# Autodesk Inventor assembly: wire_case-1
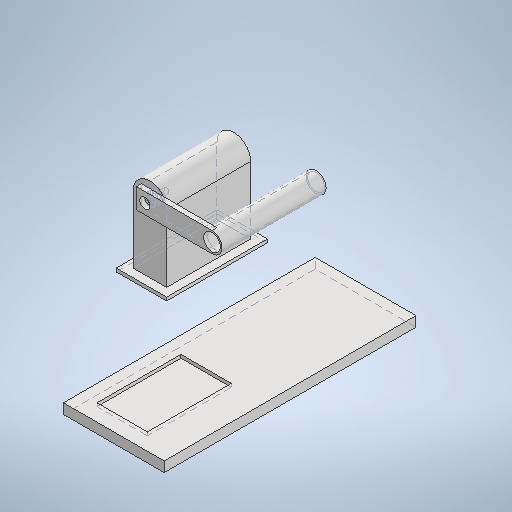
[picture p0: Inventor's stored thumbnail of the model, 512x512]
Saved by Autodesk Inventor 2025 (Build 290162000, 162)
## iProperties
Created: 2026-01-27
Part Number: wire_case-1
Document SubType Name: Assembly
Designer: mahhy
Author: mahhy
## Documents named in this file (4)
- C:\Users\mahhy\Documents\設計データ\wire_case-1\wire_case-1.iam
- C:\Users\mahhy\Documents\設計データ\wire_case-1\body-1.ipt
- C:\Users\mahhy\Documents\設計データ\wire_case-1\pole-1.ipt
- C:\Users\mahhy\Documents\設計データ\wire_case-1\body-2.ipt
## Components (3 placed, 3 different names)
1. body-1:1
2. pole-1:1 — 挿入:1
3. body-2:1 — 挿入:1
## Relationships (1: Insert 1)
- 挿入:1 [Insert]: pole-1:1 ↔ body-2:1
